# Autodesk Inventor assembly: Coluna_Suspensao_5-Cabos
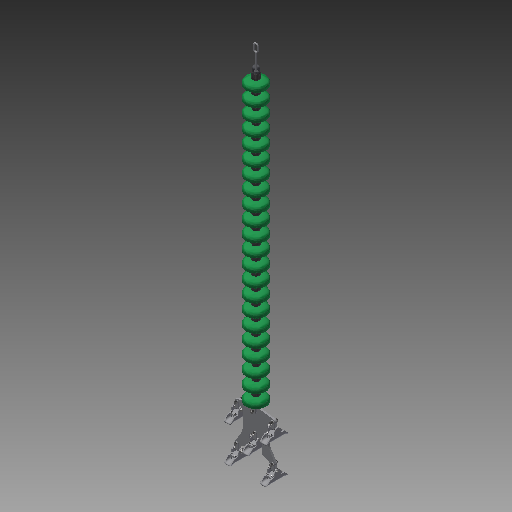
[picture p0: Inventor's stored thumbnail of the model, 512x512]
Saved by Autodesk Inventor 2018 (Build 220112000, 112)
## iProperties
Created: 2021-04-27
Part Number: Coluna_Suspensao_5-Cabos
Document SubType Name: Assembly
Designer: l01767
Author: l01767
## Documents named in this file (4)
- F:\Projetos\TAESA\Modelo 3D - Tensionadores e Suspensão\Suporte de Suspenção\Coluna_Suspensao_5-Cabos.iam
- F:\Projetos\TAESA\Modelo 3D - Tensionadores e Suspensão\Suporte de Suspenção\U300B.iam
- F:\Projetos\TAESA\Modelo 3D - Tensionadores e Suspensão\Suporte de Suspenção\Elo-Bola Longo.ipt
- F:\Projetos\TAESA\Modelo 3D - Tensionadores e Suspensão\Suporte de Suspenção\Corpo_Suspensao_Cabos.iam
## Components (46 placed, 3 different names)
1. Elo-Bola Longo:1 — Mate:1, Mate:2, Flush:4, Flush:5, Flush:6
2. Corpo_Suspensao_Cabos:1 [sub-assembly] — Mate:3, Mate:4
3. U300B:1 [sub-assembly] — Mate:2
4. U300B:2 [sub-assembly] — Mate:1
5. U300B:3 [sub-assembly]
6. U300B:4 [sub-assembly]
7. U300B:5 [sub-assembly]
8. U300B:6 [sub-assembly]
9. U300B:7 [sub-assembly]
10. U300B:8 [sub-assembly]
11. U300B:9 [sub-assembly]
12. U300B:10 [sub-assembly]
13. U300B:11 [sub-assembly]
14. U300B:12 [sub-assembly]
15. U300B:13 [sub-assembly]
16. U300B:14 [sub-assembly]
17. U300B:15 [sub-assembly]
18. U300B:16 [sub-assembly]
19. U300B:17 [sub-assembly]
20. U300B:18 [sub-assembly]
21. U300B:19 [sub-assembly]
22. U300B:20 [sub-assembly]
23. U300B:21 [sub-assembly]
24. U300B:22 [sub-assembly]
25. U300B:23 [sub-assembly]
26. U300B:24 [sub-assembly]
27. U300B:25 [sub-assembly]
28. U300B:26 [sub-assembly]
29. U300B:27 [sub-assembly]
30. U300B:28 [sub-assembly]
31. U300B:29 [sub-assembly]
32. U300B:30 [sub-assembly]
33. U300B:31 [sub-assembly]
34. U300B:32 [sub-assembly]
35. U300B:33 [sub-assembly]
36. U300B:34 [sub-assembly]
37. U300B:35 [sub-assembly]
38. U300B:36 [sub-assembly]
39. U300B:37 [sub-assembly]
40. U300B:38 [sub-assembly]
41. U300B:39 [sub-assembly]
42. U300B:40 [sub-assembly]
43. U300B:41 [sub-assembly]
44. U300B:42 [sub-assembly]
45. U300B:43 [sub-assembly]
46. U300B:44 [sub-assembly] — Mate:4
## Component patterns: (44 elements, first: U300B:1)
## Relationships (7: Mate 4, Flush 3)
- Mate:1: Elo-Bola Longo:1 ↔ U300B:2
- Mate:2: Elo-Bola Longo:1 ↔ U300B:1
- Flush:4: Elo-Bola Longo:1
- Flush:5: Elo-Bola Longo:1
- Flush:6: Elo-Bola Longo:1
- Mate:3: Corpo_Suspensao_Cabos:1
- Mate:4: Corpo_Suspensao_Cabos:1 ↔ U300B:44
